# Autodesk Inventor assembly: New Assembly
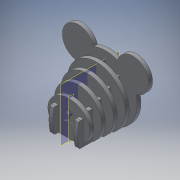
[picture p0: Inventor's stored thumbnail of the model, 180x180]
Saved by Autodesk Inventor 2019 (Build 230136000, 136)
## iProperties
Created: 2020-02-13
Part Number: New Assembly
Document SubType Name: Assembly
Designer: student
Author: student
## Documents named in this file (7)
- D:\CIM\Mini-Projects\Laser Cutter\New Assembly.iam
- D:\CIM\Mini-Projects\Laser Cutter\Head Frame.ipt
- D:\CIM\Mini-Projects\Laser Cutter\mouth.ipt
- D:\CIM\Mini-Projects\Laser Cutter\MiddlePiece1.ipt
- D:\CIM\Mini-Projects\Laser Cutter\MiddlePiece2.ipt
- D:\CIM\Mini-Projects\Laser Cutter\MiddlePiece3.ipt
- D:\CIM\Mini-Projects\Laser Cutter\BackPiece.ipt
## Components (7 placed, 6 different names)
1. Head Frame:1 — Flush:1, Flush:2, Mate:1, Mate:3, Symmetry:1
2. Head Frame:2 — Flush:1, Flush:2, Mate:1, Mate:2, Mate:4, Flush:3, Mate:5, Flush:4, Mate:7, Symmetry:1, Flush:5, Mate:9, Flush:7, Mate:10
3. mouth:1 — Mate:2, Mate:3, Mate:4, Mate:6
4. MiddlePiece1:1 — Flush:3, Mate:5, Mate:6
5. MiddlePiece2:1 — Flush:4, Mate:7, Mate:8
6. MiddlePiece3:1 — Flush:5, Flush:6, Mate:9
7. BackPiece:1 — Flush:7, Flush:8, Mate:10
## Relationships (19: Mate 10, Flush 8, Symmetry 1)
- Flush:1: Head Frame:1 ↔ Head Frame:2
- Flush:2: Head Frame:1 ↔ Head Frame:2
- Mate:1 (25.4 mm): Head Frame:1 ↔ Head Frame:2
- Mate:2: Head Frame:2 ↔ mouth:1
- Mate:3: Head Frame:1 ↔ mouth:1
- Mate:4: Head Frame:2 ↔ mouth:1
- Flush:3: Head Frame:2 ↔ MiddlePiece1:1
- Mate:5: Head Frame:2 ↔ MiddlePiece1:1
- Mate:6: mouth:1 ↔ MiddlePiece1:1
- Flush:4: Head Frame:2 ↔ MiddlePiece2:1
- Mate:7: Head Frame:2 ↔ MiddlePiece2:1
- Symmetry:1: Head Frame:1 ↔ Head Frame:2
- Mate:8: MiddlePiece2:1
- Flush:5: Head Frame:2 ↔ MiddlePiece3:1
- Flush:6: MiddlePiece3:1
- Mate:9: Head Frame:2 ↔ MiddlePiece3:1
- Flush:7: Head Frame:2 ↔ BackPiece:1
- Flush:8: BackPiece:1
- Mate:10: Head Frame:2 ↔ BackPiece:1
